# Autodesk Inventor assembly: Transmisión de correas síncronas
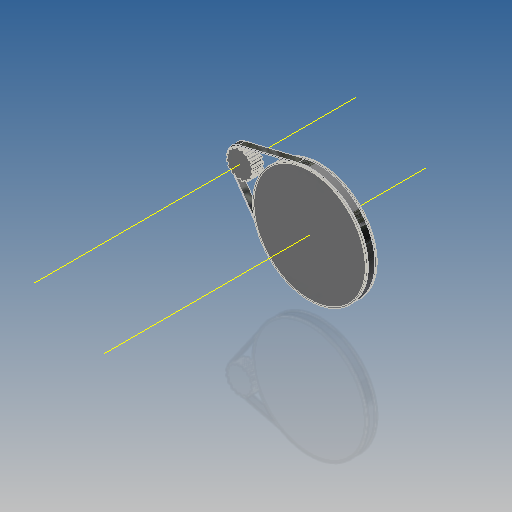
[picture p0: Inventor's stored thumbnail of the model, 512x512]
Saved by Autodesk Inventor 2017 (Build 210142000, 142)
## iProperties
ClientObjectVersion: 1
Created: 2017-03-02
Part Number: Transmisión de correas síncronas
Document SubType Name: Assembly
Designer: Leo
Author: Leo
## Documents named in this file (4)
- C:\Users\Leo\Dropbox\E\Caja Motriz\transmision Correa\Design Accelerator\Transmisión de correas síncronas1.iam
- C:\Users\Leo\Dropbox\E\Caja Motriz\transmision Correa\Design Accelerator\Correa síncrona1.ipt
- C:\Users\Leo\Dropbox\E\Caja Motriz\transmision Correa\Design Accelerator\Polea síncrona11.ipt
- C:\Users\Leo\Dropbox\E\Caja Motriz\transmision Correa\Design Accelerator\Polea síncrona21.ipt
## Components (3 placed, 3 different names)
1. Correa síncrona:1 — Nivelación:1, Coincidencia:1, Coincidencia:2, Nivelación:2, Coincidencia:3, Coincidencia:4
2. Polea síncrona1:1 — Nivelación:1, Coincidencia:1, Coincidencia:2, Rotación:1
3. Polea síncrona2:1 — Nivelación:2, Coincidencia:3, Rotación:1, Coincidencia:4
## Relationships (7: Mate 4, Flush 2, RelateRotation 1)
- Nivelación:1 [Flush]: Correa síncrona:1 ↔ Polea síncrona1:1
- Coincidencia:1 [Mate]: Correa síncrona:1 ↔ Polea síncrona1:1
- Coincidencia:2 [Mate]: Correa síncrona:1 ↔ Polea síncrona1:1
- Nivelación:2 [Flush]: Correa síncrona:1 ↔ Polea síncrona2:1
- Coincidencia:3 [Mate]: Correa síncrona:1 ↔ Polea síncrona2:1
- Rotación:1 [RelateRotation] (4 ul): Polea síncrona1:1 ↔ Polea síncrona2:1
- Coincidencia:4 [Mate]: Correa síncrona:1 ↔ Polea síncrona2:1
